# Autodesk Inventor assembly: rotor
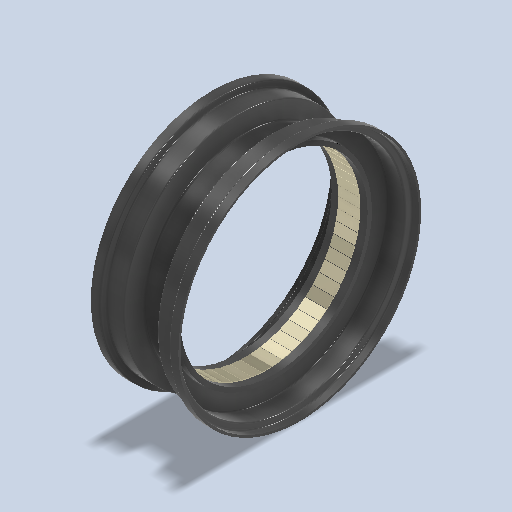
[picture p0: Inventor's stored thumbnail of the model, 512x512]
Saved by Autodesk Inventor 2026.2 (Build 302298000, 298)
## iProperties
Created: 2026-05-19
Part Number: rotor
Document SubType Name: Assembly
Designer: LENOVO
Author: LENOVO
## Documents named in this file (3)
- D:\Tugas Akhir\rotor.iam
- D:\Tugas Akhir\magnet.ipt
- D:\Tugas Akhir\velg.ipt
## Components (2 placed, 2 different names)
1. magnet:1 — Mate:1
2. velg:2 — Mate:1
## Relationships (1: Mate 1)
- Mate:1: magnet:1 ↔ velg:2
